# Autodesk Inventor assembly: testRoboRescue_Chassis_Frame
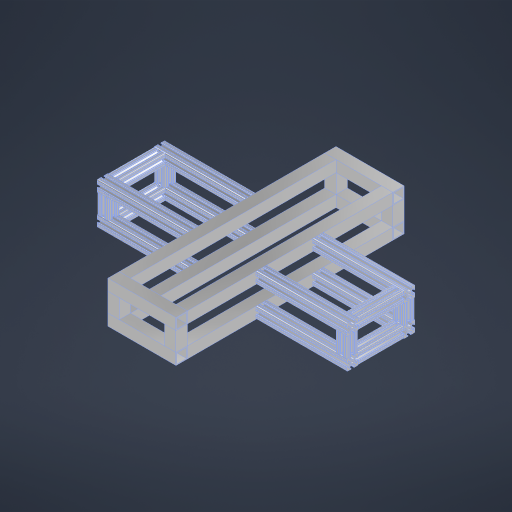
[picture p0: Inventor's stored thumbnail of the model, 512x512]
Saved by Autodesk Inventor 2023 (Build 270158000, 158)
## iProperties
Created: 2022-03-14
Part Number: testRoboRescue_Chassis_Frame
Document SubType Name: Assembly
Designer: Nebil Oumer
Author: Nebil Oumer
## Documents named in this file (5)
- E:\SBRT\testRoboRescue\Chassis\Frame\testRoboRescue_Chassis_Frame.iam
- E:\SBRT\testRoboRescue\Chassis\Frame\testRoboRescue_Chassis_Frame_heightBar.ipt
- E:\SBRT\testRoboRescue\Chassis\Frame\testRoboRescue_Chassis_Frame_widthBar.ipt
- E:\SBRT\testRoboRescue\Chassis\Frame\testRoboRescue_Chassis_Frame_lengthBar.ipt
- E:\SBRT\testRoboRescue\Chassis\Frame\8020ChassisSupport.iam
## Components (14 placed, 4 different names)
1. testRoboRescue_Chassis_Frame_heightBar:1 — Mate:4, Flush:7, Flush:8, Mate:9, Flush:18, Flush:19
2. testRoboRescue_Chassis_Frame_heightBar:2 — Mate:6, Flush:11, Flush:12, Flush:16, Flush:17, Mate:8
3. testRoboRescue_Chassis_Frame_heightBar:3 — Mate:7, Flush:13, Flush:14
4. testRoboRescue_Chassis_Frame_heightBar:4 — Flush:9, Mate:5, Flush:10, Flush:22
5. testRoboRescue_Chassis_Frame_widthBar:1 — Mate:1, Flush:1, Flush:2, Mate:2, Flush:3, Flush:4, Mate:13, Flush:26
6. testRoboRescue_Chassis_Frame_widthBar:2 — Flush:5, Mate:3, Flush:6, Flush:27
7. testRoboRescue_Chassis_Frame_widthBar:3 — Mate:10, Flush:20, Flush:21
8. testRoboRescue_Chassis_Frame_widthBar:4 — Mate:11, Flush:22, Flush:23, Mate:12
9. testRoboRescue_Chassis_Frame_lengthBar:1 — Mate:2, Flush:3, Flush:4, Flush:5, Mate:3, Flush:6, Mate:6, Flush:11, Flush:12, Mate:7, Flush:13, Flush:14, Mate:16, Angle:3
10. testRoboRescue_Chassis_Frame_lengthBar:2 — Mate:9, Flush:18, Flush:19, Mate:10, Flush:20, Flush:21, Mate:11, Flush:23
11. testRoboRescue_Chassis_Frame_lengthBar:3 — Flush:16, Flush:17, Mate:8
12. testRoboRescue_Chassis_Frame_lengthBar:4 — Mate:1, Flush:1, Flush:2, Mate:4, Flush:7, Flush:8, Flush:9, Mate:5, Flush:10, Mate:17, Angle:4, Symmetry:2
13. 8020ChassisSupport:1 [sub-assembly] — Mate:13, Flush:26, Flush:29
14. 8020ChassisSupport:2 [sub-assembly] — Mate:12, Flush:27, Mate:14, Angle:1, Mate:15, Angle:2, Flush:29
## Relationships (49: Flush 26, Mate 17, Angle 4, Symmetry 2)
- Mate:1: testRoboRescue_Chassis_Frame_widthBar:1 ↔ testRoboRescue_Chassis_Frame_lengthBar:4
- Flush:1: testRoboRescue_Chassis_Frame_widthBar:1 ↔ testRoboRescue_Chassis_Frame_lengthBar:4
- Flush:2: testRoboRescue_Chassis_Frame_widthBar:1 ↔ testRoboRescue_Chassis_Frame_lengthBar:4
- Mate:2: testRoboRescue_Chassis_Frame_widthBar:1 ↔ testRoboRescue_Chassis_Frame_lengthBar:1
- Flush:3: testRoboRescue_Chassis_Frame_widthBar:1 ↔ testRoboRescue_Chassis_Frame_lengthBar:1
- Flush:4: testRoboRescue_Chassis_Frame_widthBar:1 ↔ testRoboRescue_Chassis_Frame_lengthBar:1
- Flush:5: testRoboRescue_Chassis_Frame_widthBar:2 ↔ testRoboRescue_Chassis_Frame_lengthBar:1
- Mate:3: testRoboRescue_Chassis_Frame_widthBar:2 ↔ testRoboRescue_Chassis_Frame_lengthBar:1
- Flush:6: testRoboRescue_Chassis_Frame_widthBar:2 ↔ testRoboRescue_Chassis_Frame_lengthBar:1
- Mate:4: testRoboRescue_Chassis_Frame_heightBar:1 ↔ testRoboRescue_Chassis_Frame_lengthBar:4
- Flush:7: testRoboRescue_Chassis_Frame_heightBar:1 ↔ testRoboRescue_Chassis_Frame_lengthBar:4
- Flush:8: testRoboRescue_Chassis_Frame_heightBar:1 ↔ testRoboRescue_Chassis_Frame_lengthBar:4
- Flush:9: testRoboRescue_Chassis_Frame_heightBar:4 ↔ testRoboRescue_Chassis_Frame_lengthBar:4
- Mate:5: testRoboRescue_Chassis_Frame_heightBar:4 ↔ testRoboRescue_Chassis_Frame_lengthBar:4
- Flush:10: testRoboRescue_Chassis_Frame_heightBar:4 ↔ testRoboRescue_Chassis_Frame_lengthBar:4
- Mate:6: testRoboRescue_Chassis_Frame_heightBar:2 ↔ testRoboRescue_Chassis_Frame_lengthBar:1
- Flush:11: testRoboRescue_Chassis_Frame_heightBar:2 ↔ testRoboRescue_Chassis_Frame_lengthBar:1
- Flush:12: testRoboRescue_Chassis_Frame_heightBar:2 ↔ testRoboRescue_Chassis_Frame_lengthBar:1
- Mate:7: testRoboRescue_Chassis_Frame_heightBar:3 ↔ testRoboRescue_Chassis_Frame_lengthBar:1
- Flush:13: testRoboRescue_Chassis_Frame_heightBar:3 ↔ testRoboRescue_Chassis_Frame_lengthBar:1
- Flush:14: testRoboRescue_Chassis_Frame_heightBar:3 ↔ testRoboRescue_Chassis_Frame_lengthBar:1
- Flush:16: testRoboRescue_Chassis_Frame_heightBar:2 ↔ testRoboRescue_Chassis_Frame_lengthBar:3
- Flush:17: testRoboRescue_Chassis_Frame_heightBar:2 ↔ testRoboRescue_Chassis_Frame_lengthBar:3
- Mate:8: testRoboRescue_Chassis_Frame_heightBar:2 ↔ testRoboRescue_Chassis_Frame_lengthBar:3
- Mate:9: testRoboRescue_Chassis_Frame_heightBar:1 ↔ testRoboRescue_Chassis_Frame_lengthBar:2
- Flush:18: testRoboRescue_Chassis_Frame_heightBar:1 ↔ testRoboRescue_Chassis_Frame_lengthBar:2
- Flush:19: testRoboRescue_Chassis_Frame_heightBar:1 ↔ testRoboRescue_Chassis_Frame_lengthBar:2
- Mate:10: testRoboRescue_Chassis_Frame_widthBar:3 ↔ testRoboRescue_Chassis_Frame_lengthBar:2
- Flush:20: testRoboRescue_Chassis_Frame_widthBar:3 ↔ testRoboRescue_Chassis_Frame_lengthBar:2
- Flush:21: testRoboRescue_Chassis_Frame_widthBar:3 ↔ testRoboRescue_Chassis_Frame_lengthBar:2
- Mate:11: testRoboRescue_Chassis_Frame_widthBar:4 ↔ testRoboRescue_Chassis_Frame_lengthBar:2
- Flush:22: testRoboRescue_Chassis_Frame_heightBar:4 ↔ testRoboRescue_Chassis_Frame_widthBar:4
- Flush:23: testRoboRescue_Chassis_Frame_widthBar:4 ↔ testRoboRescue_Chassis_Frame_lengthBar:2
- Mate:12: testRoboRescue_Chassis_Frame_widthBar:4 ↔ 8020ChassisSupport:2
- Mate:13: testRoboRescue_Chassis_Frame_widthBar:1 ↔ 8020ChassisSupport:1
- Flush:26: testRoboRescue_Chassis_Frame_widthBar:1 ↔ 8020ChassisSupport:1
- Flush:27: testRoboRescue_Chassis_Frame_widthBar:2 ↔ 8020ChassisSupport:2
- Mate:14: 8020ChassisSupport:2
- Angle:1 (0 deg): 8020ChassisSupport:2
- Mate:15: 8020ChassisSupport:2
- Angle:2 (0 deg): 8020ChassisSupport:2
- Symmetry:1
- Mate:16: testRoboRescue_Chassis_Frame_lengthBar:1
- Angle:3 (0 deg): testRoboRescue_Chassis_Frame_lengthBar:1
- Mate:17: testRoboRescue_Chassis_Frame_lengthBar:4
- Angle:4 (0 deg): testRoboRescue_Chassis_Frame_lengthBar:4
- Symmetry:2: testRoboRescue_Chassis_Frame_lengthBar:4
- Flush:28
- Flush:29: 8020ChassisSupport:1 ↔ 8020ChassisSupport:2
